# Autodesk Inventor assembly: 리프트_회전부_ASSEMBLY
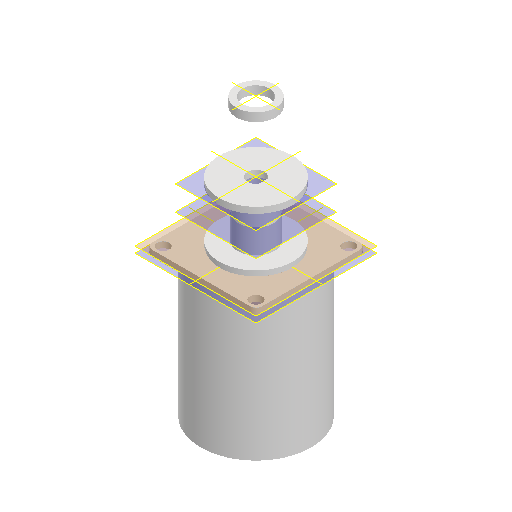
[picture p0: Inventor's stored thumbnail of the model, 512x512]
Saved by Autodesk Inventor 2027 (Build 310192000, 192)
## iProperties
Created: 2026-09-17
Part Number: 리프트_회전부_ASSEMBLY
Document SubType Name: Assembly
Designer: User
Author: User
## Documents named in this file (4)
- C:\Users\User\Desktop\4_권도영\졸업작품\INVENTOR\리프트_회전부_ASSEMBLY.iam
- C:\Users\User\Desktop\4_권도영\졸업작품\INVENTOR\모터.ipt
- C:\Users\User\Desktop\4_권도영\졸업작품\INVENTOR\도르래.ipt
- C:\Users\User\Desktop\4_권도영\졸업작품\INVENTOR\베어링.ipt
## Components (3 placed, 3 different names)
1. 모터:1 — 삽입:1
2. 도르래:2 — 삽입:1, 삽입:2
3. 베어링:1 — 삽입:2
## Relationships (2: Insert 2)
- 삽입:1 [Insert] (1 mm): 모터:1 ↔ 도르래:2
- 삽입:2 [Insert] (50 mm): 도르래:2 ↔ 베어링:1
